# Autodesk Inventor assembly: main
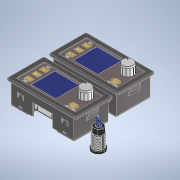
[picture p0: Inventor's stored thumbnail of the model, 180x180]
Saved by Autodesk Inventor 2022.1 (Build 261234020, 234B)
## iProperties
Created: 2022-02-06
Part Number: main
Document SubType Name: Assembly
Designer: kee
Mass: 87.5725 g
Surface Area: 681.85 cm^2
Volume: 38.129 cm^3
Density: 2.29674 g/cm^3
Author: kee
## Documents named in this file (3)
- C:\Users\logic\_workspace\2-ch-power-supply\hardware\casing\main.iam
- C:\Users\logic\_workspace\2-ch-power-supply\hardware\casing\standard_parts\DPS-5015\DPS_5015.iam
- C:\Users\logic\_workspace\2-ch-power-supply\hardware\casing\standard_parts\banana_jack\CT2236-0.iam
## Components (3 placed, 2 different names)
1. DPS_5015:1 [sub-assembly] — Flush:1, Flush:2, Mate:1
2. DPS_5015:2 [sub-assembly] — Flush:1, Flush:2, Mate:1
3. CT2236-black:1 [sub-assembly]
## Relationships (3: Flush 2, Mate 1)
- Flush:1: DPS_5015:1 ↔ DPS_5015:2
- Flush:2: DPS_5015:1 ↔ DPS_5015:2
- Mate:1 (5 mm): DPS_5015:1 ↔ DPS_5015:2
